# Autodesk Inventor assembly: GE-13024
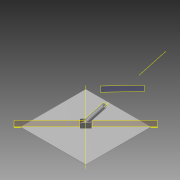
[picture p0: Inventor's stored thumbnail of the model, 180x180]
Saved by Autodesk Inventor 2013 (Build 170138000, 138)
## iProperties
Created: 2013-01-06
Part Number: GE-13024
Document SubType Name: Assembly
Designer: Phillip
Author: Phillip
## Documents named in this file (3)
- E:\Data Folder\FIRST 2013\FIRST KOP\FIRST Arena 2013\Pyramid\GE-13024.iam
- E:\Data Folder\FIRST 2013\FIRST KOP\FIRST Arena 2013\Pyramid\GE-13025.iam
- E:\Data Folder\FIRST 2013\FIRST KOP\FIRST Arena 2013\Pyramid\GE-13026.iam
## Components (2 placed, 2 different names)
1. GE-13025:1 [sub-assembly] — Mate:1, Mate:4, Angle:2, Mate:7, Angle:3
2. GE-13026:1 [sub-assembly] — Mate:1, Mate:2, Angle:1, Mate:6, Angle:3
## Relationships (11: Mate 8, Angle 3)
- Mate:1: GE-13025:1 ↔ GE-13026:1
- Mate:2: GE-13026:1
- Mate:3
- Angle:1 (0 deg): GE-13026:1
- Mate:4: GE-13025:1
- Angle:2 (0 deg): GE-13025:1
- Mate:5
- Mate:6: GE-13026:1
- Mate:7: GE-13025:1
- Mate:8
- Angle:3 (60 deg): GE-13025:1 ↔ GE-13026:1
